# Autodesk Inventor assembly: Horquilla
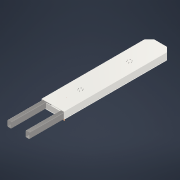
[picture p0: Inventor's stored thumbnail of the model, 180x180]
Saved by Autodesk Inventor 2022 (Build 260153000, 153)
## iProperties
Created: 2021-09-10
Part Number: Horquilla
Document SubType Name: Assembly
Designer: seb_0
Author: seb_0
## Documents named in this file (7)
- D:\Documentos\15.PUCP_2021-2\[PDM] Proyecto de Diseño Mecatrónico\ProyectoGIT\ProyectoRobotPallet\Horquillas\Horquilla.iam
- D:\Documentos\15.PUCP_2021-2\[PDM] Proyecto de Diseño Mecatrónico\ProyectoGIT\ProyectoRobotPallet\Horquillas\Horquilla_Base.ipt
- D:\Documentos\15.PUCP_2021-2\[PDM] Proyecto de Diseño Mecatrónico\ProyectoGIT\ProyectoRobotPallet\Horquillas\Horquilla_Cubierta.ipt
- D:\Documentos\15.PUCP_2021-2\[PDM] Proyecto de Diseño Mecatrónico\ProyectoGIT\ProyectoRobotPallet\Horquillas\Rueda_Soporte.ipt
- D:\Documentos\15.PUCP_2021-2\[PDM] Proyecto de Diseño Mecatrónico\ProyectoGIT\ProyectoRobotPallet\Horquillas\Rueda_Rueda.ipt
- D:\Documentos\15.PUCP_2021-2\[PDM] Proyecto de Diseño Mecatrónico\ProyectoGIT\ProyectoRobotPallet\Horquillas\DIN 59 410 - 60x40x2.9-1400.ipt
- D:\Documentos\15.PUCP_2021-2\[PDM] Proyecto de Diseño Mecatrónico\ProyectoGIT\ProyectoRobotPallet\SistemaDeElevación\SistemaDeElevación.iam
## Components (8 placed, 6 different names)
1. Horquilla_Base:1 — Coincidencia:1, Coincidencia:2, Coincidencia:3, Nivelación:1, Nivelación:2, Coincidencia:4, Coincidencia:15, Coincidencia:17, Coincidencia:18, Nivelación:5, Nivelación:6, Nivelación:7, Nivelación:8, Coincidencia:19, Mate:20, Mate:24
2. Horquilla_Cubierta:1 — Nivelación:1, Nivelación:2, Coincidencia:19, Mate:22, Mate:25
3. Rueda_Soporte:1 — Coincidencia:4, Coincidencia:5, Coincidencia:15
4. Rueda_Rueda:1 — Coincidencia:5
5. DIN 59 410 - 60x40x2.9-1400:1 — Coincidencia:18, Nivelación:5, Nivelación:8, Mate:21, Flush:9, Mate:23
6. DIN 59 410 - 60x40x2.9-1400:2 — Coincidencia:17, Nivelación:6, Nivelación:7
7. SistemaDeElevación:1 [sub-assembly] — Mate:20, Mate:21, Mate:22, Flush:9, Flush:10
8. SistemaDeElevación:2 [sub-assembly] — Mate:23, Mate:24, Flush:10, Mate:25
## Relationships (23: Mate 15, Flush 8)
- Coincidencia:1 [Mate]: Horquilla_Base:1
- Coincidencia:2 [Mate]: Horquilla_Base:1
- Coincidencia:3 [Mate]: Horquilla_Base:1
- Nivelación:1 [Flush]: Horquilla_Base:1 ↔ Horquilla_Cubierta:1
- Nivelación:2 [Flush]: Horquilla_Base:1 ↔ Horquilla_Cubierta:1
- Coincidencia:4 [Mate]: Horquilla_Base:1 ↔ Rueda_Soporte:1
- Coincidencia:5 [Mate]: Rueda_Soporte:1 ↔ Rueda_Rueda:1
- Coincidencia:15 [Mate]: Horquilla_Base:1 ↔ Rueda_Soporte:1
- Coincidencia:17 [Mate]: Horquilla_Base:1 ↔ DIN 59 410 - 60x40x2.9-1400:2
- Coincidencia:18 [Mate]: Horquilla_Base:1 ↔ DIN 59 410 - 60x40x2.9-1400:1
- Nivelación:5 [Flush] (2.5 mm): Horquilla_Base:1 ↔ DIN 59 410 - 60x40x2.9-1400:1
- Nivelación:6 [Flush] (2.5 mm): Horquilla_Base:1 ↔ DIN 59 410 - 60x40x2.9-1400:2
- Nivelación:7 [Flush] (50 mm): Horquilla_Base:1 ↔ DIN 59 410 - 60x40x2.9-1400:2
- Nivelación:8 [Flush] (50 mm): Horquilla_Base:1 ↔ DIN 59 410 - 60x40x2.9-1400:1
- Coincidencia:19 [Mate]: Horquilla_Base:1 ↔ Horquilla_Cubierta:1
- Mate:20: Horquilla_Base:1 ↔ SistemaDeElevación:1
- Mate:21: DIN 59 410 - 60x40x2.9-1400:1 ↔ SistemaDeElevación:1
- Mate:22: Horquilla_Cubierta:1 ↔ SistemaDeElevación:1
- Flush:9 (200 mm): DIN 59 410 - 60x40x2.9-1400:1 ↔ SistemaDeElevación:1
- Mate:23: DIN 59 410 - 60x40x2.9-1400:1 ↔ SistemaDeElevación:2
- Mate:24: Horquilla_Base:1 ↔ SistemaDeElevación:2
- Flush:10 (500 mm): SistemaDeElevación:1 ↔ SistemaDeElevación:2
- Mate:25: Horquilla_Cubierta:1 ↔ SistemaDeElevación:2
